# Autodesk Inventor assembly: Leg_joint_roll_pitch
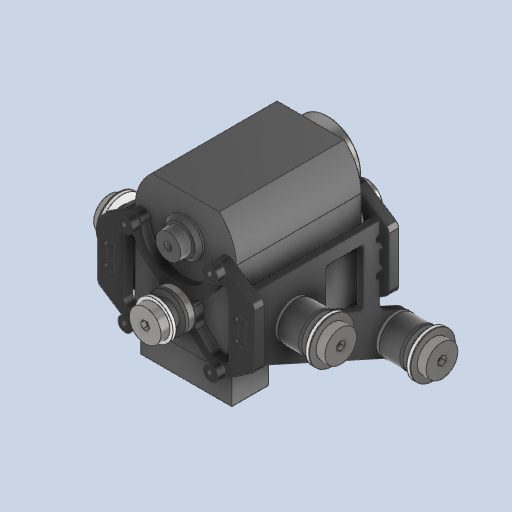
[picture p0: Inventor's stored thumbnail of the model, 512x512]
Saved by Autodesk Inventor 2022.3 (Build 263350000, 350)
## iProperties
Created: 2022-06-15
Part Number: Leg_joint_roll_pitch
Document SubType Name: Assembly
Designer: Masato Kubotera
Mass: 129.389 g
Surface Area: 379.222 cm^2
Volume: 74.7337 cm^3
Density: 1.73133 g/cm^3
Author: Masato Kubotera
## Documents named in this file (21)
- C:\Users\Masato\Desktop\SUSTAINA-OP\LowerBody\Leg_joint\Leg_joint_roll_pitch.iam
- C:\Users\Masato\Desktop\SUSTAINA-OP\LowerBody\Leg_joint\Leg_joint_pitch_frame.ipt
- C:\Users\Masato\Desktop\SUSTAINA-OP\LowerBody\Leg_joint\Leg_joint_roll_frame.ipt
- C:\Users\Masato\Desktop\SUSTAINA-OP\ReadyMade\KONDO\B3M-SC-1170-A_with_ClampHorn.iam
- C:\Users\Masato\Desktop\SUSTAINA-OP\ReadyMade\InsertNut\S4-05-3W.ipt
- C:\Users\Masato\Desktop\SUSTAINA-OP\ReadyMade\InsertNut\SF419.ipt
- C:\Users\Masato\Desktop\SUSTAINA-OP\ReadyMade\Spacer\ABLSBF6-39.5-M4-N4.ipt
- C:\Users\Masato\Desktop\SUSTAINA-OP\ReadyMade\Washer\UUW-0412-10H.ipt
- C:\Users\Masato\Desktop\SUSTAINA-OP\ReadyMade\Washer\CCC-0612-65B.ipt
- C:\Users\Masato\Desktop\SUSTAINA-OP\ReadyMade\Bush\80F-0603.ipt
- C:\Users\Masato\Desktop\SUSTAINA-OP\ReadyMade\Screw\DBTS4-11-6-DHC.ipt
- C:\Users\Masato\Desktop\SUSTAINA-OP\ReadyMade\Screw\DBTS4-11-8-DHC.ipt
- C:\Users\Masato\Desktop\SUSTAINA-OP\ReadyMade\Screw\DBTS4-5-5-DHC.ipt
- C:\Users\Masato\Desktop\SUSTAINA-OP\ReadyMade\Washer\UUW-0412-20H.ipt
- C:\Users\Masato\Desktop\SUSTAINA-OP\ReadyMade\Washer\CC-0612-50B.ipt
- C:\Users\Masato\Desktop\SUSTAINA-OP\ReadyMade\Washer\TT-0612-10.ipt
- C:\Users\Masato\Desktop\SUSTAINA-OP\ReadyMade\Washer\TT-0814-10.ipt
- C:\Users\Masato\Desktop\SUSTAINA-OP\ReadyMade\Washer\UUW-0614-03H.ipt
- C:\Users\Masato\Desktop\SUSTAINA-OP\ReadyMade\Screw\FC-2620EB.ipt
- C:\Users\Masato\Desktop\SUSTAINA-OP\ReadyMade\Screw\FC-2615EB.ipt
- C:\Users\Masato\Desktop\SUSTAINA-OP\ReadyMade\Screw\DBTS4-10-5-DHC.ipt
## Components (49 placed, 20 different names)
1. DBTS4-10-5-DHC:1 — Insert:56, Insert:57
2. UUW-0412-20H:2 — Insert:54, Insert:55, Insert:56
3. Leg_joint_pitch_frame:1 — 挿入:1, メイト:3, メイト:4, フラッシュ:2, フラッシュ:3, 挿入:13, 挿入:15, 挿入:16
4. Leg_joint_roll_frame:1 — 挿入:3, 角度:1, 挿入:5, 挿入:6, 挿入:7, 挿入:8, メイト:3, メイト:4, フラッシュ:2, メイト:5, メイト:6, 挿入:31, 挿入:48, 挿入:49, 挿入:50, 挿入:51
5. Leg_joint_pitch_frame:2 — 挿入:2, メイト:5, メイト:6, フラッシュ:3, 挿入:14, 挿入:17, 挿入:18
6. Leg_joint_roll_frame:2 — 挿入:4, 角度:2, 挿入:9, 挿入:10, 挿入:11, 挿入:12, 挿入:52, 挿入:53, Insert:54
7. ABLSBF6-39.5-M4-N4:1 — 挿入:13, 挿入:14
8. UUW-0412-10H:1 — 挿入:15, 挿入:19, 挿入:27
9. UUW-0412-10H:2 — 挿入:16, 挿入:20, 挿入:29
10. UUW-0412-10H:3 — 挿入:17, 挿入:21, 挿入:28
11. UUW-0412-10H:4 — 挿入:18, 挿入:22, 挿入:30
12. CCC-0612-65B:1 — 挿入:19, 挿入:23
13. CCC-0612-65B:2 — 挿入:20, 挿入:24
14. CCC-0612-65B:3 — 挿入:21, 挿入:25
15. CCC-0612-65B:4 — 挿入:22, 挿入:26
16. 80F-0603:1 — 挿入:23
17. 80F-0603:2 — 挿入:24
18. 80F-0603:3 — 挿入:25
19. 80F-0603:4 — 挿入:26
20. B3M-SC-1170-A_with_ClampHorn:1 [sub-assembly] — メイト:1, メイト:2, フラッシュ:1, 挿入:5, 挿入:6, 挿入:7, 挿入:8, 挿入:9, 挿入:10, 挿入:11, 挿入:12
21. S4-05-3W:1 — 挿入:3, 角度:1
22. SF419:1 — 挿入:1
23. S4-05-3W:2 — 挿入:4, 角度:2
24. SF419:2 — 挿入:2
25. UUW-0412-20H:1 — 挿入:31, 挿入:34, 挿入:36
26. CC-0612-50B:1 — 挿入:35, Insert:55
27. 80F-0603:5 — 挿入:34
28. 80F-0603:6 — 挿入:35
29. TT-0612-10:1 — 挿入:38
30. TT-0612-10:2 — Insert:57
31. TT-0814-10:1 — 挿入:42
32. UUW-0614-03H:1 — 挿入:40, 挿入:42
33. TT-0814-10:2 — 挿入:43
34. UUW-0614-03H:2 — 挿入:41, 挿入:43
35. TT-0814-10:3 — 挿入:46
36. UUW-0614-03H:3 — 挿入:44, 挿入:46
37. TT-0814-10:4 — 挿入:47
38. UUW-0614-03H:4 — 挿入:45, 挿入:47
39. FC-2620EB:1 — 挿入:48
40. FC-2620EB:2 — 挿入:49
41. FC-2620EB:3 — 挿入:50
42. FC-2620EB:4 — 挿入:51
43. FC-2615EB:1 — 挿入:52
44. FC-2615EB:2 — 挿入:53
45. DBTS4-11-6-DHC:1 — 挿入:27, 挿入:40
46. DBTS4-11-6-DHC:2 — 挿入:28, 挿入:41
47. DBTS4-11-8-DHC:1 — 挿入:29, 挿入:44
48. DBTS4-11-8-DHC:2 — 挿入:30, 挿入:45
49. DBTS4-5-5-DHC:1 — 挿入:36, 挿入:38
## Relationships (64: Insert 53, Mate 6, Flush 3, Angle 2)
- メイト:1 [Mate]: B3M-SC-1170-A_with_ClampHorn:1
- メイト:2 [Mate]: B3M-SC-1170-A_with_ClampHorn:1
- フラッシュ:1 [Flush]: B3M-SC-1170-A_with_ClampHorn:1
- 挿入:1 [Insert]: Leg_joint_pitch_frame:1 ↔ SF419:1
- 挿入:2 [Insert]: Leg_joint_pitch_frame:2 ↔ SF419:2
- 挿入:3 [Insert]: Leg_joint_roll_frame:1 ↔ S4-05-3W:1
- 挿入:4 [Insert]: Leg_joint_roll_frame:2 ↔ S4-05-3W:2
- 角度:1 [Angle] (0 deg): Leg_joint_roll_frame:1 ↔ S4-05-3W:1
- 角度:2 [Angle] (0 deg): Leg_joint_roll_frame:2 ↔ S4-05-3W:2
- 挿入:5 [Insert]: Leg_joint_roll_frame:1 ↔ B3M-SC-1170-A_with_ClampHorn:1
- 挿入:6 [Insert]: Leg_joint_roll_frame:1 ↔ B3M-SC-1170-A_with_ClampHorn:1
- 挿入:7 [Insert]: Leg_joint_roll_frame:1 ↔ B3M-SC-1170-A_with_ClampHorn:1
- 挿入:8 [Insert]: Leg_joint_roll_frame:1 ↔ B3M-SC-1170-A_with_ClampHorn:1
- 挿入:9 [Insert]: Leg_joint_roll_frame:2 ↔ B3M-SC-1170-A_with_ClampHorn:1
- 挿入:10 [Insert]: Leg_joint_roll_frame:2 ↔ B3M-SC-1170-A_with_ClampHorn:1
- 挿入:11 [Insert]: Leg_joint_roll_frame:2 ↔ B3M-SC-1170-A_with_ClampHorn:1
- 挿入:12 [Insert]: Leg_joint_roll_frame:2 ↔ B3M-SC-1170-A_with_ClampHorn:1
- メイト:3 [Mate] (0.025 mm): Leg_joint_pitch_frame:1 ↔ Leg_joint_roll_frame:1
- メイト:4 [Mate] (0.025 mm): Leg_joint_pitch_frame:1 ↔ Leg_joint_roll_frame:1
- フラッシュ:2 [Flush]: Leg_joint_pitch_frame:1 ↔ Leg_joint_roll_frame:1
- メイト:5 [Mate] (0.025 mm): Leg_joint_roll_frame:1 ↔ Leg_joint_pitch_frame:2
- メイト:6 [Mate] (0.025 mm): Leg_joint_roll_frame:1 ↔ Leg_joint_pitch_frame:2
- フラッシュ:3 [Flush]: Leg_joint_pitch_frame:1 ↔ Leg_joint_pitch_frame:2
- 挿入:13 [Insert]: Leg_joint_pitch_frame:1 ↔ ABLSBF6-39.5-M4-N4:1
- 挿入:14 [Insert]: Leg_joint_pitch_frame:2 ↔ ABLSBF6-39.5-M4-N4:1
- 挿入:15 [Insert]: Leg_joint_pitch_frame:1 ↔ UUW-0412-10H:1
- 挿入:16 [Insert]: Leg_joint_pitch_frame:1 ↔ UUW-0412-10H:2
- 挿入:17 [Insert]: Leg_joint_pitch_frame:2 ↔ UUW-0412-10H:3
- 挿入:18 [Insert]: Leg_joint_pitch_frame:2 ↔ UUW-0412-10H:4
- 挿入:19 [Insert]: UUW-0412-10H:1 ↔ CCC-0612-65B:1
- 挿入:20 [Insert]: UUW-0412-10H:2 ↔ CCC-0612-65B:2
- 挿入:21 [Insert]: UUW-0412-10H:3 ↔ CCC-0612-65B:3
- 挿入:22 [Insert]: UUW-0412-10H:4 ↔ CCC-0612-65B:4
- 挿入:23 [Insert]: CCC-0612-65B:1 ↔ 80F-0603:1
- 挿入:24 [Insert]: CCC-0612-65B:2 ↔ 80F-0603:2
- 挿入:25 [Insert]: CCC-0612-65B:3 ↔ 80F-0603:3
- 挿入:26 [Insert]: CCC-0612-65B:4 ↔ 80F-0603:4
- 挿入:27 [Insert]: UUW-0412-10H:1 ↔ DBTS4-11-6-DHC:1
- 挿入:28 [Insert]: UUW-0412-10H:3 ↔ DBTS4-11-6-DHC:2
- 挿入:29 [Insert]: UUW-0412-10H:2 ↔ DBTS4-11-8-DHC:1
- 挿入:30 [Insert]: UUW-0412-10H:4 ↔ DBTS4-11-8-DHC:2
- 挿入:31 [Insert]: Leg_joint_roll_frame:1 ↔ UUW-0412-20H:1
- 挿入:34 [Insert]: UUW-0412-20H:1 ↔ 80F-0603:5
- 挿入:35 [Insert]: CC-0612-50B:1 ↔ 80F-0603:6
- 挿入:36 [Insert]: UUW-0412-20H:1 ↔ DBTS4-5-5-DHC:1
- 挿入:38 [Insert]: TT-0612-10:1 ↔ DBTS4-5-5-DHC:1
- 挿入:40 [Insert]: UUW-0614-03H:1 ↔ DBTS4-11-6-DHC:1
- 挿入:41 [Insert]: UUW-0614-03H:2 ↔ DBTS4-11-6-DHC:2
- 挿入:42 [Insert]: TT-0814-10:1 ↔ UUW-0614-03H:1
- 挿入:43 [Insert]: TT-0814-10:2 ↔ UUW-0614-03H:2
- 挿入:44 [Insert]: UUW-0614-03H:3 ↔ DBTS4-11-8-DHC:1
- 挿入:45 [Insert]: UUW-0614-03H:4 ↔ DBTS4-11-8-DHC:2
- 挿入:46 [Insert]: TT-0814-10:3 ↔ UUW-0614-03H:3
- 挿入:47 [Insert]: TT-0814-10:4 ↔ UUW-0614-03H:4
- 挿入:48 [Insert]: Leg_joint_roll_frame:1 ↔ FC-2620EB:1
- 挿入:49 [Insert]: Leg_joint_roll_frame:1 ↔ FC-2620EB:2
- 挿入:50 [Insert]: Leg_joint_roll_frame:1 ↔ FC-2620EB:3
- 挿入:51 [Insert]: Leg_joint_roll_frame:1 ↔ FC-2620EB:4
- 挿入:52 [Insert]: Leg_joint_roll_frame:2 ↔ FC-2615EB:1
- 挿入:53 [Insert]: Leg_joint_roll_frame:2 ↔ FC-2615EB:2
- Insert:54: UUW-0412-20H:2 ↔ Leg_joint_roll_frame:2
- Insert:55: UUW-0412-20H:2 ↔ CC-0612-50B:1
- Insert:56: DBTS4-10-5-DHC:1 ↔ UUW-0412-20H:2
- Insert:57: DBTS4-10-5-DHC:1 ↔ TT-0612-10:2
